# Autodesk Inventor assembly: ShooterPrototype-ver4-1111-2021
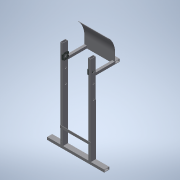
[picture p0: Inventor's stored thumbnail of the model, 180x180]
Saved by Autodesk Inventor 2021 (Build 250183000, 183)
## iProperties
Created: 2020-01-17
Part Number: ShooterPrototype-ver4-1111-2021
Document SubType Name: Assembly
Designer: JMHal
Author: JMHal
## Documents named in this file (8)
- F:\PHRC CADD 2021\PHRC CADD\2020 Infinite Recharge\Shooting\Assemblies\ShooterPrototype-ver4-1111-2021.iam
- F:\PHRC CADD 2021\PHRC CADD\2020 Infinite Recharge\Shooting\Parts\12in 2x1 Aluminum Block-ver1-1111-2019.ipt
- F:\PHRC CADD 2021\PHRC CADD\2020 Infinite Recharge\Shooting\Parts\16in 2x1 Aluminum Block-ver1-1111-2019.ipt
- F:\PHRC CADD 2021\PHRC CADD\2020 Infinite Recharge\Shooting\Parts\12in Aluminum Plate-ver-1-1111-2019.ipt
- F:\PHRC CADD 2021\PHRC CADD\2020 Infinite Recharge\Shooting\Parts\VersaBlock-ver1-1111-2019.ipt
- F:\PHRC CADD 2021\PHRC CADD\2020 Infinite Recharge\Shooting\Parts\ShooterBracketHorizontal.ver1-1111-2020.ipt
- F:\PHRC CADD 2021\PHRC CADD\2020 Infinite Recharge\Shooting\Parts\Hood.ver1-1111-2020.ipt
- F:\PHRC CADD 2021\PHRC CADD\2020 Infinite Recharge\Shooting\Parts\ShooterBracket.ver2-1111-2021.ipt
## Components (10 placed, 7 different names)
1. 12in 2x1 Aluminum Block-ver1-1111-2019:1 — Mate:22, Flush:5, Flush:6, Flush:7, Flush:18, Flush:20
2. 12in Aluminum Plate-ver-1-1111-2019:1 — Mate:12, Mate:13, Flush:2
3. 16in 2x1 Aluminum Block-ver1-1111-2019:3 — Mate:12, Mate:13, Angle:3, Flush:4, Flush:7, Symmetry:1, Mate:31, Flush:19, Angle:5
4. 16in 2x1 Aluminum Block-ver1-1111-2019:4 — Angle:4, Flush:2, Flush:4, Mate:22, Flush:5, Flush:6, Symmetry:1, Mate:30, Flush:17, Flush:25
5. VersaBlock-ver1-1111-2019:3 — Angle:3
6. VersaBlock-ver1-1111-2019:4 — Angle:4
7. ShooterBracketHorizontal.ver1-1111-2020:1 — Mate:33, Flush:23, Flush:24
8. Hood.ver1-1111-2020:1 — Mate:32, Flush:21, Flush:22, Mate:33, Flush:23, Flush:24
9. ShooterBracket.ver2-1111-2021:1 — Mate:30, Flush:17, Flush:18, Mate:32, Flush:21, Flush:22
10. ShooterBracket.ver2-1111-2021:2 — Mate:31, Flush:19, Flush:20
## Relationships (26: Flush 15, Mate 7, Angle 3, Symmetry 1)
- Mate:12: 12in Aluminum Plate-ver-1-1111-2019:1 ↔ 16in 2x1 Aluminum Block-ver1-1111-2019:3
- Mate:13: 12in Aluminum Plate-ver-1-1111-2019:1 ↔ 16in 2x1 Aluminum Block-ver1-1111-2019:3
- Angle:3 (0 deg): 16in 2x1 Aluminum Block-ver1-1111-2019:3 ↔ VersaBlock-ver1-1111-2019:3
- Angle:4 (0 deg): 16in 2x1 Aluminum Block-ver1-1111-2019:4 ↔ VersaBlock-ver1-1111-2019:4
- Flush:2: 12in Aluminum Plate-ver-1-1111-2019:1 ↔ 16in 2x1 Aluminum Block-ver1-1111-2019:4
- Flush:4: 16in 2x1 Aluminum Block-ver1-1111-2019:3 ↔ 16in 2x1 Aluminum Block-ver1-1111-2019:4
- Mate:22: 12in 2x1 Aluminum Block-ver1-1111-2019:1 ↔ 16in 2x1 Aluminum Block-ver1-1111-2019:4
- Flush:5: 12in 2x1 Aluminum Block-ver1-1111-2019:1 ↔ 16in 2x1 Aluminum Block-ver1-1111-2019:4
- Flush:6 (-133.35 mm): 12in 2x1 Aluminum Block-ver1-1111-2019:1 ↔ 16in 2x1 Aluminum Block-ver1-1111-2019:4
- Flush:7: 12in 2x1 Aluminum Block-ver1-1111-2019:1 ↔ 16in 2x1 Aluminum Block-ver1-1111-2019:3
- Symmetry:1: 16in 2x1 Aluminum Block-ver1-1111-2019:3 ↔ 16in 2x1 Aluminum Block-ver1-1111-2019:4
- Mate:30: 16in 2x1 Aluminum Block-ver1-1111-2019:4 ↔ ShooterBracket.ver2-1111-2021:1
- Flush:17: 16in 2x1 Aluminum Block-ver1-1111-2019:4 ↔ ShooterBracket.ver2-1111-2021:1
- Flush:18 (-749.3 mm): 12in 2x1 Aluminum Block-ver1-1111-2019:1 ↔ ShooterBracket.ver2-1111-2021:1
- Mate:31: 16in 2x1 Aluminum Block-ver1-1111-2019:3 ↔ ShooterBracket.ver2-1111-2021:2
- Flush:19: 16in 2x1 Aluminum Block-ver1-1111-2019:3 ↔ ShooterBracket.ver2-1111-2021:2
- Flush:20 (-749.3 mm): 12in 2x1 Aluminum Block-ver1-1111-2019:1 ↔ ShooterBracket.ver2-1111-2021:2
- Mate:32: Hood.ver1-1111-2020:1 ↔ ShooterBracket.ver2-1111-2021:1
- Flush:21: Hood.ver1-1111-2020:1 ↔ ShooterBracket.ver2-1111-2021:1
- Flush:22: Hood.ver1-1111-2020:1 ↔ ShooterBracket.ver2-1111-2021:1
- Mate:33: ShooterBracketHorizontal.ver1-1111-2020:1 ↔ Hood.ver1-1111-2020:1
- Flush:23: ShooterBracketHorizontal.ver1-1111-2020:1 ↔ Hood.ver1-1111-2020:1
- Flush:24: ShooterBracketHorizontal.ver1-1111-2020:1 ↔ Hood.ver1-1111-2020:1
- Flush:25 (1.778 mm): 16in 2x1 Aluminum Block-ver1-1111-2019:4
- Angle:5 (0 deg): 16in 2x1 Aluminum Block-ver1-1111-2019:3
- Flush:26 (8.89 mm)
